# Autodesk Inventor assembly: Auspressrolle_befaesstigung
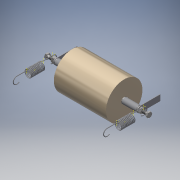
[picture p0: Inventor's stored thumbnail of the model, 180x180]
Saved by Autodesk Inventor 2018 (Build 220112000, 112)
## iProperties
Created: 2018-01-12
Part Number: Auspressrolle_befaesstigung
Material: Generisch
Document SubType Name: Assembly
Designer: Julian
Author: Julian
## Documents named in this file (9)
- C:\Users\Julian\Desktop\Schule\5AHME\Diplomarbeit\Git\fuettr_prototype\Mechanical\Inventorskizzen\Auspressrolle_befaesstigung.iam
- C:\Users\Julian\Desktop\Schule\5AHME\Diplomarbeit\Git\fuettr_prototype\Mechanical\Inventorskizzen\Auspressrolle.ipt
- C:\Users\Julian\Desktop\Schule\5AHME\Diplomarbeit\Git\fuettr_prototype\Mechanical\Inventorskizzen\Verbindungsstück_Rolle.ipt
- C:\Users\Julian\Desktop\Schule\5AHME\Diplomarbeit\Git\fuettr_prototype\Mechanical\Inventorskizzen\Kunststoffrolle_antrieb.ipt
- C:\Users\Julian\Documents\Inventor\Content Center Files\R2018\de-DE\DIN 471(1)\DIN 471 - 8x0,8.ipt
- C:\Users\Julian\Documents\Inventor\Content Center Files\R2018\de-DE\ISO 4017(1)\ISO 4017 - M5 x 25 - ISO.ipt
- C:\Users\Julian\Documents\Inventor\Content Center Files\R2018\de-DE\ISO 4032(2)\ISO 4032 - M5 - ISO.ipt
- C:\Users\Julian\Documents\Inventor\Content Center Files\R2018\de-DE\ISO 7090\ISO 7090 - 5 - 140 HV(1).ipt
- C:\Users\Julian\Desktop\Schule\5AHME\Diplomarbeit\Git\fuettr_prototype\Mechanical\Inventorskizzen\Feder.ipt
## Components (16 placed, 8 different names)
1. Auspressrolle:1 — Passend:1, Fluchtend:1, Starr:4, Starr:3, Drehbar:1, Drehbar:3
2. Kunststoffrolle_antrieb:1 — Passend:1, Fluchtend:1
3. DIN 471 8x0,8:1 — Starr:3
4. DIN 471 8x0,8:2 — Starr:4
5. ISO 4017 M5 x 25:1 — Starr:6
6. ISO 4017 M5 x 25:2 — Starr:5
7. ISO 4032 M5:1 — Drehbar:7, Drehbar:10
8. ISO 4032 M5:2 — Drehbar:8, Drehbar:9
9. ISO 7090 5 - 140 HV:1 — Drehbar:1, Drehbar:2
10. ISO 7090 5 - 140 HV:2 — Drehbar:6, Starr:6, Drehbar:7
11. ISO 7090 5 - 140 HV:3 — Drehbar:3, Drehbar:4
12. ISO 7090 5 - 140 HV:4 — Drehbar:5, Starr:5, Drehbar:8
13. Verbindungsstück_Rolle:1 — Drehbar:2, Drehbar:6
14. Verbindungsstück_Rolle:2 — Drehbar:4, Drehbar:5
15. Feder:1 — Drehbar:9
16. Feder:2 — Drehbar:10
## Relationships (16: RevoluteJoint 10, WeldJoint 4, Mate 1, Flush 1)
- Passend:1 [Mate]: Auspressrolle:1 ↔ Kunststoffrolle_antrieb:1
- Fluchtend:1 [Flush]: Auspressrolle:1 ↔ Kunststoffrolle_antrieb:1
- Starr:4 [WeldJoint]: Auspressrolle:1 ↔ DIN 471 8x0,8:2
- Starr:3 [WeldJoint]: Auspressrolle:1 ↔ DIN 471 8x0,8:1
- Drehbar:1 [RevoluteJoint]: Auspressrolle:1 ↔ ISO 7090 5 - 140 HV:1
- Drehbar:2 [RevoluteJoint]: ISO 7090 5 - 140 HV:1 ↔ Verbindungsstück_Rolle:1
- Drehbar:3 [RevoluteJoint]: Auspressrolle:1 ↔ ISO 7090 5 - 140 HV:3
- Drehbar:4 [RevoluteJoint]: ISO 7090 5 - 140 HV:3 ↔ Verbindungsstück_Rolle:2
- Drehbar:5 [RevoluteJoint]: ISO 7090 5 - 140 HV:4 ↔ Verbindungsstück_Rolle:2
- Starr:5 [WeldJoint]: ISO 4017 M5 x 25:2 ↔ ISO 7090 5 - 140 HV:4
- Drehbar:6 [RevoluteJoint]: ISO 7090 5 - 140 HV:2 ↔ Verbindungsstück_Rolle:1
- Starr:6 [WeldJoint]: ISO 4017 M5 x 25:1 ↔ ISO 7090 5 - 140 HV:2
- Drehbar:7 [RevoluteJoint]: ISO 4032 M5:1 ↔ ISO 7090 5 - 140 HV:2
- Drehbar:8 [RevoluteJoint]: ISO 4032 M5:2 ↔ ISO 7090 5 - 140 HV:4
- Drehbar:9 [RevoluteJoint]: ISO 4032 M5:2 ↔ Feder:1
- Drehbar:10 [RevoluteJoint]: ISO 4032 M5:1 ↔ Feder:2
